# Autodesk Inventor assembly: TalonSRX_SparkMAX_Tower_Assy
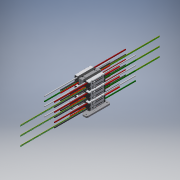
[picture p0: Inventor's stored thumbnail of the model, 180x180]
Saved by Autodesk Inventor 2018.3 (Build 223284000, 284)
## iProperties
Created: 2019-01-19
Part Number: TalonSRX_SparkMAX_Tower_Assy
Document SubType Name: Assembly
Designer: kopytn
Author: kopytn
## Documents named in this file (4)
- C:\Users\kopytn\Desktop\5030 CAD\Talon SRX Tower\TalonSRX_SparkMAX_Tower_Assy.iam
- C:\Users\kopytn\Desktop\5030 CAD\Talon SRX Tower\TalonSRX_SparkMAX_Tower-2019A.ipt
- C:\Users\kopytn\Desktop\5030 CAD\Talon SRX Tower\REV-11-2158.ipt
- C:\Users\kopytn\Desktop\5030 CAD\Talon SRX Tower\Talon_SRX_217-8080.ipt
## Components (13 placed, 3 different names)
1. TalonSRX_SparkMAX_Tower-2019A:1 — Mate:1, Flush:1, Mate:2, Mate:3, Mate:4, Mate:5, Mate:7, Mate:8, Mate:9, Mate:10
2. REV-11-2158:2 — Mate:5, Mate:6, Flush:2
3. REV-11-2158:1 — Mate:3, Mate:4, Mate:6, Flush:2
4. REV-11-2158:3
5. REV-11-2158:4
6. REV-11-2158:5
7. REV-11-2158:6
8. Talon_SRX_217-8080:2 — Mate:9, Mate:10, Mate:11
9. Talon_SRX_217-8080:1 — Mate:7, Mate:8, Mate:11
10. Talon_SRX_217-8080:3
11. Talon_SRX_217-8080:4
12. Talon_SRX_217-8080:5
13. Talon_SRX_217-8080:6
## Component patterns: (3 elements, first: REV-11-2158:2 + REV-11-2158:1), (3 elements, first: Talon_SRX_217-8080:2 + Talon_SRX_217-8080:1)
## Relationships (13: Mate 11, Flush 2)
- Mate:1: TalonSRX_SparkMAX_Tower-2019A:1
- Flush:1: TalonSRX_SparkMAX_Tower-2019A:1
- Mate:2: TalonSRX_SparkMAX_Tower-2019A:1
- Mate:3: TalonSRX_SparkMAX_Tower-2019A:1 ↔ REV-11-2158:1
- Mate:4: TalonSRX_SparkMAX_Tower-2019A:1 ↔ REV-11-2158:1
- Mate:5: TalonSRX_SparkMAX_Tower-2019A:1 ↔ REV-11-2158:2
- Mate:6: REV-11-2158:2 ↔ REV-11-2158:1
- Flush:2: REV-11-2158:2 ↔ REV-11-2158:1
- Mate:7: TalonSRX_SparkMAX_Tower-2019A:1 ↔ Talon_SRX_217-8080:1
- Mate:8: TalonSRX_SparkMAX_Tower-2019A:1 ↔ Talon_SRX_217-8080:1
- Mate:9: TalonSRX_SparkMAX_Tower-2019A:1 ↔ Talon_SRX_217-8080:2
- Mate:10: TalonSRX_SparkMAX_Tower-2019A:1 ↔ Talon_SRX_217-8080:2
- Mate:11: Talon_SRX_217-8080:2 ↔ Talon_SRX_217-8080:1
